# Autodesk Inventor assembly: Chuck Assembly
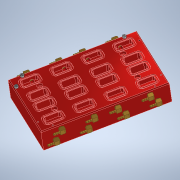
[picture p0: Inventor's stored thumbnail of the model, 180x180]
Saved by Autodesk Inventor 2022 (Build 260153000, 153)
## iProperties
Created: 2021-01-11
Part Number: Chuck Assembly
Document SubType Name: Assembly
Designer: caleb
Author: caleb
## Documents named in this file (4)
- C:\Users\Caleb\Desktop\nebraska-silicon-lab\Hardware\ETL\Module Assembly\Chuck - 16-pocket V1\Chuck - 16-pocket.iam
- C:\Users\Caleb\Desktop\nebraska-silicon-lab\Hardware\ETL\Module Assembly\Chuck - 16-pocket V1\90128A212_ZNC-PLTD ALLOY STL SCKT HEAD CAP SCREW.ipt
- C:\Users\Caleb\Desktop\nebraska-silicon-lab\Hardware\ETL\Module Assembly\Chuck - 16-pocket V1\44555K147_BRASS BARBED TUBE FITTING FOR VACUUM.ipt
- C:\Users\Caleb\Desktop\nebraska-silicon-lab\Hardware\ETL\Module Assembly\Chuck - 16-pocket V1\Chuck - 16-pocket.ipt
## Components (20 placed, 3 different names)
1. Chuck - 16-pocket:1 — Insert:1, Insert:2, Insert:3, Insert:4, Insert:5, Insert:6, Insert:7, Insert:8, Insert:9, Insert:10, Insert:11, Insert:12, Insert:13, Insert:14, Insert:15, Insert:16, Insert:17, Insert:18, Insert:19, Angle:1, Angle:2, Angle:3, Angle:4, Angle:5, Angle:6, Angle:7, Angle:8, Angle:9, Angle:10, Angle:11, Angle:12, Angle:13, Angle:14, Angle:15, Angle:16
2. 90128A212_ZNC-PLTD ALLOY STL SCKT HEAD CAP SCREW:1 — Insert:2
3. 90128A212_ZNC-PLTD ALLOY STL SCKT HEAD CAP SCREW:2 — Insert:3
4. 90128A212_ZNC-PLTD ALLOY STL SCKT HEAD CAP SCREW:3 — Insert:1
5. 44555K147_BRASS BARBED TUBE FITTING FOR VACUUM:1 — Insert:4, Angle:9
6. 44555K147_BRASS BARBED TUBE FITTING FOR VACUUM:2 — Insert:5, Angle:10
7. 44555K147_BRASS BARBED TUBE FITTING FOR VACUUM:3 — Insert:7, Angle:12
8. 44555K147_BRASS BARBED TUBE FITTING FOR VACUUM:4 — Insert:6, Angle:11
9. 44555K147_BRASS BARBED TUBE FITTING FOR VACUUM:5 — Insert:9, Angle:14
10. 44555K147_BRASS BARBED TUBE FITTING FOR VACUUM:6 — Insert:8, Angle:13
11. 44555K147_BRASS BARBED TUBE FITTING FOR VACUUM:7 — Insert:10, Angle:16
12. 44555K147_BRASS BARBED TUBE FITTING FOR VACUUM:8 — Insert:11, Angle:15
13. 44555K147_BRASS BARBED TUBE FITTING FOR VACUUM:9 — Insert:12, Angle:1
14. 44555K147_BRASS BARBED TUBE FITTING FOR VACUUM:10 — Insert:13, Angle:2
15. 44555K147_BRASS BARBED TUBE FITTING FOR VACUUM:11 — Insert:14, Angle:4
16. 44555K147_BRASS BARBED TUBE FITTING FOR VACUUM:12 — Insert:15, Angle:3
17. 44555K147_BRASS BARBED TUBE FITTING FOR VACUUM:13 — Insert:16, Angle:6
18. 44555K147_BRASS BARBED TUBE FITTING FOR VACUUM:14 — Insert:17, Angle:5
19. 44555K147_BRASS BARBED TUBE FITTING FOR VACUUM:15 — Insert:18, Angle:8
20. 44555K147_BRASS BARBED TUBE FITTING FOR VACUUM:16 — Insert:19, Angle:7
## Relationships (35: Insert 19, Angle 16)
- Insert:1: Chuck - 16-pocket:1 ↔ 90128A212_ZNC-PLTD ALLOY STL SCKT HEAD CAP SCREW:3
- Insert:2: Chuck - 16-pocket:1 ↔ 90128A212_ZNC-PLTD ALLOY STL SCKT HEAD CAP SCREW:1
- Insert:3: Chuck - 16-pocket:1 ↔ 90128A212_ZNC-PLTD ALLOY STL SCKT HEAD CAP SCREW:2
- Insert:4: Chuck - 16-pocket:1 ↔ 44555K147_BRASS BARBED TUBE FITTING FOR VACUUM:1
- Insert:5: Chuck - 16-pocket:1 ↔ 44555K147_BRASS BARBED TUBE FITTING FOR VACUUM:2
- Insert:6: Chuck - 16-pocket:1 ↔ 44555K147_BRASS BARBED TUBE FITTING FOR VACUUM:4
- Insert:7: Chuck - 16-pocket:1 ↔ 44555K147_BRASS BARBED TUBE FITTING FOR VACUUM:3
- Insert:8: Chuck - 16-pocket:1 ↔ 44555K147_BRASS BARBED TUBE FITTING FOR VACUUM:6
- Insert:9: Chuck - 16-pocket:1 ↔ 44555K147_BRASS BARBED TUBE FITTING FOR VACUUM:5
- Insert:10: Chuck - 16-pocket:1 ↔ 44555K147_BRASS BARBED TUBE FITTING FOR VACUUM:7
- Insert:11: Chuck - 16-pocket:1 ↔ 44555K147_BRASS BARBED TUBE FITTING FOR VACUUM:8
- Insert:12: Chuck - 16-pocket:1 ↔ 44555K147_BRASS BARBED TUBE FITTING FOR VACUUM:9
- Insert:13: Chuck - 16-pocket:1 ↔ 44555K147_BRASS BARBED TUBE FITTING FOR VACUUM:10
- Insert:14: Chuck - 16-pocket:1 ↔ 44555K147_BRASS BARBED TUBE FITTING FOR VACUUM:11
- Insert:15: Chuck - 16-pocket:1 ↔ 44555K147_BRASS BARBED TUBE FITTING FOR VACUUM:12
- Insert:16: Chuck - 16-pocket:1 ↔ 44555K147_BRASS BARBED TUBE FITTING FOR VACUUM:13
- Insert:17: Chuck - 16-pocket:1 ↔ 44555K147_BRASS BARBED TUBE FITTING FOR VACUUM:14
- Insert:18: Chuck - 16-pocket:1 ↔ 44555K147_BRASS BARBED TUBE FITTING FOR VACUUM:15
- Insert:19: Chuck - 16-pocket:1 ↔ 44555K147_BRASS BARBED TUBE FITTING FOR VACUUM:16
- Angle:1 (0 deg): Chuck - 16-pocket:1 ↔ 44555K147_BRASS BARBED TUBE FITTING FOR VACUUM:9
- Angle:2 (0 deg): Chuck - 16-pocket:1 ↔ 44555K147_BRASS BARBED TUBE FITTING FOR VACUUM:10
- Angle:3 (0 deg): Chuck - 16-pocket:1 ↔ 44555K147_BRASS BARBED TUBE FITTING FOR VACUUM:12
- Angle:4 (0 deg): Chuck - 16-pocket:1 ↔ 44555K147_BRASS BARBED TUBE FITTING FOR VACUUM:11
- Angle:5 (0 deg): Chuck - 16-pocket:1 ↔ 44555K147_BRASS BARBED TUBE FITTING FOR VACUUM:14
- Angle:6 (0 deg): Chuck - 16-pocket:1 ↔ 44555K147_BRASS BARBED TUBE FITTING FOR VACUUM:13
- Angle:7 (0 deg): Chuck - 16-pocket:1 ↔ 44555K147_BRASS BARBED TUBE FITTING FOR VACUUM:16
- Angle:8 (0 deg): Chuck - 16-pocket:1 ↔ 44555K147_BRASS BARBED TUBE FITTING FOR VACUUM:15
- Angle:9 (0 deg): Chuck - 16-pocket:1 ↔ 44555K147_BRASS BARBED TUBE FITTING FOR VACUUM:1
- Angle:10 (0 deg): Chuck - 16-pocket:1 ↔ 44555K147_BRASS BARBED TUBE FITTING FOR VACUUM:2
- Angle:11 (0 deg): Chuck - 16-pocket:1 ↔ 44555K147_BRASS BARBED TUBE FITTING FOR VACUUM:4
- Angle:12 (0 deg): Chuck - 16-pocket:1 ↔ 44555K147_BRASS BARBED TUBE FITTING FOR VACUUM:3
- Angle:13 (0 deg): Chuck - 16-pocket:1 ↔ 44555K147_BRASS BARBED TUBE FITTING FOR VACUUM:6
- Angle:14 (0 deg): Chuck - 16-pocket:1 ↔ 44555K147_BRASS BARBED TUBE FITTING FOR VACUUM:5
- Angle:15 (0 deg): Chuck - 16-pocket:1 ↔ 44555K147_BRASS BARBED TUBE FITTING FOR VACUUM:8
- Angle:16 (0 deg): Chuck - 16-pocket:1 ↔ 44555K147_BRASS BARBED TUBE FITTING FOR VACUUM:7
